# Autodesk Inventor assembly: 知能ロボコン発射台３.1
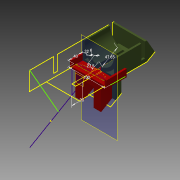
[picture p0: Inventor's stored thumbnail of the model, 180x180]
Saved by Autodesk Inventor 2013 (Build 170138000, 138)
## iProperties
Created: 2014-05-17
Part Number: 知能ロボコン発射台３.1
Document SubType Name: Assembly
Designer: horumo136
Mass: 518.958 g
Surface Area: 1361.17 cm^2
Volume: 489.583 cm^3
Density: 1.06 g/cm^3
Author: horumo136
## Documents named in this file (3)
- C:\Users\horumo136\Documents\知能ロボコン発射台３.1.iam
- C:\Users\horumo136\Documents\知能ロボコン発射台２.ipt
- C:\Users\horumo136\Documents\知能ロボコン発射台支え.ipt
## Components (2 placed, 2 different names)
1. 知能ロボコン発射台２:1 — メイト:1, メイト:2, メイト:3
2. 知能ロボコン発射台支え:1 — メイト:1, メイト:2, メイト:3
## Relationships (3: Mate 3)
- メイト:1 [Mate]: 知能ロボコン発射台２:1 ↔ 知能ロボコン発射台支え:1
- メイト:2 [Mate]: 知能ロボコン発射台２:1 ↔ 知能ロボコン発射台支え:1
- メイト:3 [Mate]: 知能ロボコン発射台２:1 ↔ 知能ロボコン発射台支え:1
